# Autodesk Inventor assembly: Epsilon intake
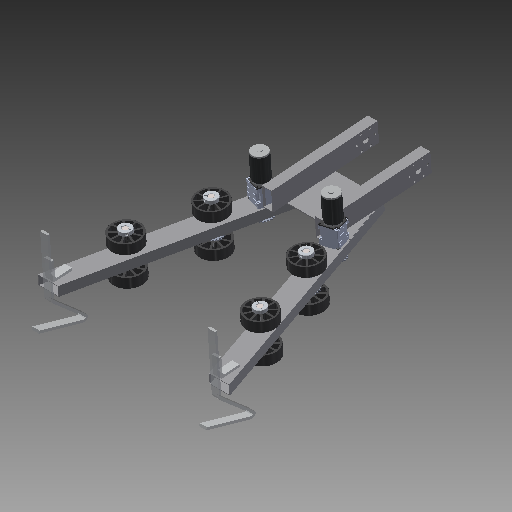
[picture p0: Inventor's stored thumbnail of the model, 512x512]
Saved by Autodesk Inventor 2019 (Build 230136000, 136)
## iProperties
Created: 2019-02-18
Part Number: Epsilon intake
Document SubType Name: Assembly
Designer: josh
Mass: 1477.37 g
Surface Area: 10570.1 cm^2
Volume: 1477.37 cm^3
Density: 1 g/cm^3
Author: josh
## Documents named in this file (7)
- D:\Synthesis Robots\Epsilon\Epsilon Grabbers\Epsilon intake.iam
- D:\Synthesis Robots\Epsilon\Epsilon Grabbers\Aluminum grabber mount.ipt
- D:\Synthesis Robots\Epsilon\Epsilon Grabbers\Trapezoid support plate.ipt
- D:\Synthesis Robots\Epsilon\Epsilon Grabbers\Epsilon Grabbers.iam
- D:\Synthesis Robots\Epsilon\Epsilon Grabbers\Epsilon grabbers 2.iam
- D:\Synthesis Robots\Epsilon\Epsilon Grabbers\Plexi disc mount.ipt
- D:\Synthesis Robots\Epsilon\Plexi intake\Plexi hooks.ipt
## Components (9 placed, 6 different names)
1. Aluminum grabber mount:1
2. Aluminum grabber mount:2
3. Trapezoid support plate:1 — Mate:7, Mate:8, Flush:6
4. Epsilon Grabbers:1 [sub-assembly] — Mate:9, Flush:7
5. Epsilon grabbers 2:1 [sub-assembly] — Mate:7, Mate:8, Flush:6, Mate:10, Flush:9
6. Plexi disc mount:1 — Mate:9, Flush:7, Flush:8
7. Plexi disc mount:2 — Mate:10, Flush:9, Mate:11, Flush:10
8. Plexi hooks:1 — Flush:8, Flush:11
9. Plexi hooks:2 — Mate:11, Flush:10, Flush:11
## Relationships (19: Flush 10, Mate 9)
- [Flush]: Aluminum grabber mount:1 ↔ Aluminum grabber mount:2
- [Flush]: Aluminum grabber mount:1 ↔ Aluminum grabber mount:2
- [Mate]: Aluminum grabber mount:2 ↔ Trapezoid support plate:1
- [Flush] (38.1 mm): Aluminum grabber mount:2 ↔ Trapezoid support plate:1
- [Mate]: Aluminum grabber mount:1 ↔ Trapezoid support plate:1
- [Mate]: Trapezoid support plate:1 ↔ Epsilon Grabbers:1
- [Flush]: Trapezoid support plate:1 ↔ Epsilon Grabbers:1
- [Mate]: Trapezoid support plate:1 ↔ Epsilon Grabbers:1
- Mate:7: Trapezoid support plate:1 ↔ Epsilon grabbers 2:1
- Mate:8: Trapezoid support plate:1 ↔ Epsilon grabbers 2:1
- Flush:6: Trapezoid support plate:1 ↔ Epsilon grabbers 2:1
- Mate:9: Epsilon Grabbers:1 ↔ Plexi disc mount:1
- Flush:7: Epsilon Grabbers:1 ↔ Plexi disc mount:1
- Flush:8: Plexi disc mount:1 ↔ Plexi hooks:1
- Mate:10: Epsilon grabbers 2:1 ↔ Plexi disc mount:2
- Flush:9: Epsilon grabbers 2:1 ↔ Plexi disc mount:2
- Mate:11: Plexi disc mount:2 ↔ Plexi hooks:2
- Flush:10: Plexi disc mount:2 ↔ Plexi hooks:2
- Flush:11: Plexi hooks:1 ↔ Plexi hooks:2
